# Autodesk Inventor assembly: ForkMount
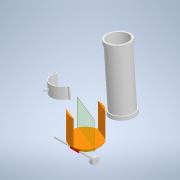
[picture p0: Inventor's stored thumbnail of the model, 180x180]
Saved by Autodesk Inventor 2021 (Build 250183000, 183)
## iProperties
Created: 2020-05-25
Part Number: ForkMount
Document SubType Name: Assembly
Designer: robst
Author: robst
## Documents named in this file (8)
- C:\git\CAD-Development\robSteele\ShapeWays\TelescopeProjects\TelescopeMount\ForkMount.iam
- C:\git\CAD-Development\robSteele\ShapeWays\TelescopeProjects\TelescopeMount\baseV01.ipt
- C:\git\CAD-Development\robSteele\ShapeWays\TelescopeProjects\TelescopeMount\ForkMount\Design Accelerator\Worm Gears2.iam
- C:\git\CAD-Development\robSteele\ShapeWays\TelescopeProjects\TelescopeMount\raHandController.ipt
- C:\git\CAD-Development\robSteele\ShapeWays\TelescopeProjects\TelescopeMount\12x3_8-keyedDriveShaft.ipt
- C:\git\CAD-Development\robSteele\ShapeWays\TelescopeProjects\TelescopeMount\topOfRaBase.ipt
- C:\git\CAD-Development\robSteele\ShapeWays\TelescopeProjects\TelescopeMount\tubeBracket.ipt
- C:\git\CAD-Development\robSteele\ShapeWays\TelescopeProjects\TelescopeMount\telescopeTube.ipt
## Components (7 placed, 7 different names)
1. baseV01:1 — Mate:1, Mate:2
2. Worm Gears:1 [sub-assembly] — Mate:1, Mate:2, Mate:3, Mate:4, Insert:2
3. 12x3_8-keyedDriveShaft:1 — Mate:3, Mate:4, Flush:1
4. raHandController:1 — Flush:1
5. topOfRaBase:1 — Insert:2
6. tubeBracket:1
7. telescopeTube:1
## Relationships (6: Mate 4, Flush 1, Insert 1)
- Mate:1: baseV01:1 ↔ Worm Gears:1
- Mate:2 (19.05 mm): baseV01:1 ↔ Worm Gears:1
- Mate:3: Worm Gears:1 ↔ 12x3_8-keyedDriveShaft:1
- Mate:4: Worm Gears:1 ↔ 12x3_8-keyedDriveShaft:1
- Flush:1: 12x3_8-keyedDriveShaft:1 ↔ raHandController:1
- Insert:2 (19.05 mm): Worm Gears:1 ↔ topOfRaBase:1
